# Autodesk Inventor assembly: GE-09031
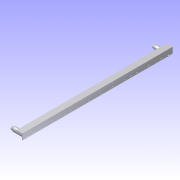
[picture p0: Inventor's stored thumbnail of the model, 180x180]
Saved by Autodesk Inventor 2012 (Build 160160000, 160)
## iProperties
Created: 2008-05-27
Part Number: GE-09031
Description: Top Rail - Corner
Document SubType Name: Assembly
Designer: dfoster
Title: Top Rail - Corner
Author: narosenberg
## Documents named in this file (4)
- C:\Data Folder\FRC 2012 Field\Components\GE-09031.iam
- C:\Data Folder\FRC 2012 Field\Components\GE-09031-01.ipt
- C:\Data Folder\FRC 2012 Field\Components\GE-09031-02.ipt
- C:\Data Folder\FRC 2012 Field\Components\GE-09031-03.ipt
## Components (4 placed, 3 different names)
1. GE-09031-01:1 — Mate:1, Flush:1, Flush:2
2. GE-09031-02:1 — Mate:1, Flush:1, Flush:2
3. GE-09031-03:1
4. GE-09031-03:2
## Relationships (5: Flush 2, Insert 2, Mate 1)
- Mate:1: GE-09031-01:1 ↔ GE-09031-02:1
- Flush:1 (-1.5875 mm): GE-09031-01:1 ↔ GE-09031-02:1
- Flush:2 (-74.6125 mm): GE-09031-01:1 ↔ GE-09031-02:1
- [Insert]: GE-09031-01:1 ↔ GE-09031-03:2
- [Insert]: GE-09031-01:1 ↔ GE-09031-03:1
